# Autodesk Inventor assembly: Motor_Bar
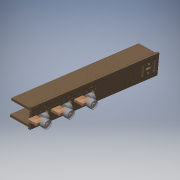
[picture p0: Inventor's stored thumbnail of the model, 180x180]
Saved by Autodesk Inventor 2016 (Build 200138000, 138)
## iProperties
Created: 2016-01-06
Part Number: Motor_Bar
Document SubType Name: Assembly
Designer: m2memari
Author: m2memari
## Documents named in this file (5)
- C:\MoDonGD\Jane\ShadowGame\ShadowGame\Motor_Bar.iam
- C:\MoDonGD\Jane\ShadowGame\ShadowGame\BearingMotorColumn.ipt
- C:\MoDonGD\Jane\ShadowGame\ShadowGame\BearingMotorColumnSupport.ipt
- C:\MoDonGD\Jane\ShadowGame\ShadowGame\BearingStand_V2.ipt
- C:\MoDonGD\Jane\ShadowGame\ShadowGame\Bearing.ipt
## Components (12 placed, 4 different names)
1. BearingMotorColumn:1 — Mate:1, Mate:2, Mate:3, Mate:4, Mate:5, Mate:6, Mate:7, Mate:8, Mate:9, Mate:10, Mate:11, Mate:12, Mate:13, Mate:14, Mate:15
2. BearingMotorColumnSupport:1 — Mate:1, Mate:2, Mate:3
3. BearingMotorColumnSupport:2 — Mate:4, Mate:5, Mate:6
4. BearingStand_V2:1 — Mate:9, Mate:12, Mate:15, Mate:19, Mate:21, Tangent:5, Tangent:6, Tangent:9, Tangent:10
5. BearingStand_V2:2 — Mate:8, Mate:11, Mate:14, Mate:18, Mate:20, Tangent:7, Tangent:8, Tangent:11, Tangent:12
6. BearingStand_V2:3 — Mate:7, Mate:10, Mate:13, Tangent:1, Mate:16, Tangent:2, Mate:17, Tangent:3, Tangent:4
7. Bearing:1 — Mate:17, Tangent:3, Tangent:4
8. Bearing:2 — Mate:20, Tangent:7, Tangent:8
9. Bearing:3 — Mate:21, Tangent:5, Tangent:6
10. Bearing:4 — Tangent:1, Mate:16, Tangent:2
11. Bearing:5 — Mate:19, Tangent:9, Tangent:10
12. Bearing:6 — Mate:18, Tangent:11, Tangent:12
## Relationships (33: Mate 21, Tangent 12)
- Mate:1: BearingMotorColumn:1 ↔ BearingMotorColumnSupport:1
- Mate:2: BearingMotorColumn:1 ↔ BearingMotorColumnSupport:1
- Mate:3: BearingMotorColumn:1 ↔ BearingMotorColumnSupport:1
- Mate:4: BearingMotorColumn:1 ↔ BearingMotorColumnSupport:2
- Mate:5: BearingMotorColumn:1 ↔ BearingMotorColumnSupport:2
- Mate:6: BearingMotorColumn:1 ↔ BearingMotorColumnSupport:2
- Mate:7: BearingMotorColumn:1 ↔ BearingStand_V2:3
- Mate:8: BearingMotorColumn:1 ↔ BearingStand_V2:2
- Mate:9: BearingMotorColumn:1 ↔ BearingStand_V2:1
- Mate:10: BearingMotorColumn:1 ↔ BearingStand_V2:3
- Mate:11: BearingMotorColumn:1 ↔ BearingStand_V2:2
- Mate:12: BearingMotorColumn:1 ↔ BearingStand_V2:1
- Mate:13: BearingMotorColumn:1 ↔ BearingStand_V2:3
- Mate:14: BearingMotorColumn:1 ↔ BearingStand_V2:2
- Mate:15: BearingMotorColumn:1 ↔ BearingStand_V2:1
- Tangent:1: BearingStand_V2:3 ↔ Bearing:4
- Mate:16: BearingStand_V2:3 ↔ Bearing:4
- Tangent:2: BearingStand_V2:3 ↔ Bearing:4
- Mate:17: BearingStand_V2:3 ↔ Bearing:1
- Tangent:3: BearingStand_V2:3 ↔ Bearing:1
- Tangent:4: BearingStand_V2:3 ↔ Bearing:1
- Mate:18: BearingStand_V2:2 ↔ Bearing:6
- Mate:19: BearingStand_V2:1 ↔ Bearing:5
- Mate:20: BearingStand_V2:2 ↔ Bearing:2
- Mate:21: BearingStand_V2:1 ↔ Bearing:3
- Tangent:5: BearingStand_V2:1 ↔ Bearing:3
- Tangent:6: BearingStand_V2:1 ↔ Bearing:3
- Tangent:7: BearingStand_V2:2 ↔ Bearing:2
- Tangent:8: BearingStand_V2:2 ↔ Bearing:2
- Tangent:9: BearingStand_V2:1 ↔ Bearing:5
- Tangent:10: BearingStand_V2:1 ↔ Bearing:5
- Tangent:11: BearingStand_V2:2 ↔ Bearing:6
- Tangent:12: BearingStand_V2:2 ↔ Bearing:6
